# Autodesk Inventor assembly: Zespół1
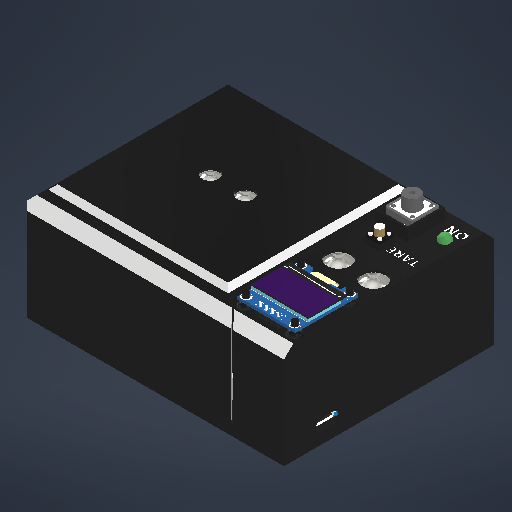
[picture p0: Inventor's stored thumbnail of the model, 512x512]
Saved by Autodesk Inventor 2027 (Build 310192060, 192F)
## iProperties
Created: 2026-03-26
Part Number: Zespół1
Document SubType Name: Assembly
Designer: User
Author: User
## Documents named in this file (16)
- G:\Github\Scale\Hardware\Model\Zespół1.iam
- G:\Github\Scale\Hardware\Model\taca.ipt
- G:\Github\Scale\Hardware\Model\bridz.ipt
- G:\Github\Scale\Hardware\Model\klappa.ipt
- G:\Github\Scale\Hardware\Model\TP4056_Charging_Module_Type_C\TP4056_Charging_Module_Type_C\TP4056_Charging_Module_Type_C.ipt
- G:\Github\Scale\Hardware\Model\GUZIK.ipt
- G:\Github\Scale\Hardware\Model\92000A328_Passivated 18-8 Stainless Steel Pan Head Phillips Screws\92000A328_Passivated 18-8 Stainless Steel Pan Head Phillips Screws\92000A328_Passivated 18-8 Stainle.ipt
- G:\Github\Scale\Hardware\Model\92000A220_Passivated 18-8 Stainless Steel Pan Head Phillips Screws\92000A220_Passivated 18-8 Stainless Steel Pan Head Phillips Screws\92000A220_Passivated 18-8 Stainle.ipt
- G:\Github\Scale\Hardware\Model\mypushbutton\mypushbutton\mypushbutton.ipt
- G:\Github\Scale\Hardware\Model\JesusMC_led 5mm v1\JesusMC_led 5mm v1\JesusMC_led 5mm v1.ipt
- G:\Github\Scale\Hardware\Model\0.96'' OLED Display\0.96'' OLED Display.ipt
- G:\Github\Scale\Hardware\Model\LoadCell-20kg-80mm\LoadCell-20kg-80mm.ipt
- G:\Github\Scale\Hardware\Model\Zespół1\AIP\FEA\fhv00ujy8.fins
- G:\Github\Scale\Hardware\Model\Zespół1\AIP\FEA\fhv00uk1s.fsat
- G:\Github\Scale\Hardware\Model\Zespół1\AIP\FEA\fhv00uk2o.ftes
- G:\Github\Scale\Hardware\Model\Zespół1\AIP\FEA\fhv00uk2o.fwiz
## Components (13 placed, 11 different names)
1. taca:1 — Obrotowe:8, Sztywne:6
2. bridz:1 — Sztywne:1, Sztywne:2, Zestawiające:2, Zestawiające:3, Zestawiające:4, Obrotowe:11
3. klappa:1 — Sztywne:1, Obrotowe:6, Obrotowe:7, Sztywne:4, Sztywne:5, Obrotowe:9, Obrotowe:10
4. TP4056_Charging_Module_Type_C:1 — Sztywne:2
5. GUZIK:1 — Obrotowe:6
6. mypushbutton:1 — Sztywne:4
7. JesusMC_led 5mm v1:1 — Sztywne:5
8. 0.96'' OLED Display:1 — Obrotowe:9, Obrotowe:10
9. LoadCell-20kg-80mm:1 — Obrotowe:11, Sztywne:6
10. 92000A328_Passivated 18-8 Stainle:1 — Obrotowe:7
11. 92000A328_Passivated 18-8 Stainle:2
12. 92000A220_Passivated 18-8 Stainle:1 — Obrotowe:8
13. 92000A220_Passivated 18-8 Stainle:2
## Component patterns: (2 elements, first: 92000A328_Passivated 18-8 Stainle:1), (2 elements, first: 92000A220_Passivated 18-8 Stainle:1)
## Relationships (14: RevoluteJoint 6, WeldJoint 5, Mate 3)
- Sztywne:1 [WeldJoint] (12.7 mm): bridz:1 ↔ klappa:1
- Sztywne:2 [WeldJoint] (0.4 mm): bridz:1 ↔ TP4056_Charging_Module_Type_C:1
- Obrotowe:6 [RevoluteJoint] (-2 mm): klappa:1 ↔ GUZIK:1
- Obrotowe:7 [RevoluteJoint] (-21 mm): klappa:1 ↔ 92000A328_Passivated 18-8 Stainle:1
- Obrotowe:8 [RevoluteJoint] (-10 mm): taca:1 ↔ 92000A220_Passivated 18-8 Stainle:1
- Sztywne:4 [WeldJoint]: klappa:1 ↔ mypushbutton:1
- Zestawiające:2 [Mate]: bridz:1
- Zestawiające:3 [Mate]: bridz:1
- Zestawiające:4 [Mate]: bridz:1
- Sztywne:5 [WeldJoint]: klappa:1 ↔ JesusMC_led 5mm v1:1
- Obrotowe:9 [RevoluteJoint]: klappa:1 ↔ 0.96'' OLED Display:1
- Obrotowe:10 [RevoluteJoint]: klappa:1 ↔ 0.96'' OLED Display:1
- Obrotowe:11 [RevoluteJoint]: bridz:1 ↔ LoadCell-20kg-80mm:1
- Sztywne:6 [WeldJoint]: taca:1 ↔ LoadCell-20kg-80mm:1
